# Autodesk Inventor assembly: cable-hanger-hook
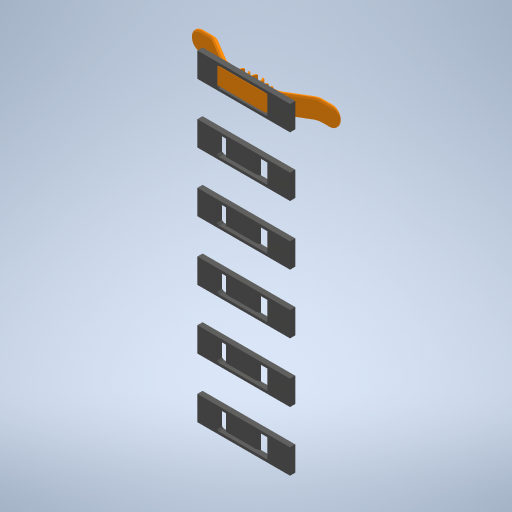
[picture p0: Inventor's stored thumbnail of the model, 512x512]
Saved by Autodesk Inventor 2023 (Build 270158030, 158C)
## iProperties
Created: 2024-09-23
Part Number: cable-hanger-hook
Document SubType Name: Assembly
Designer: Imogen Heard
Author: Imogen Heard
## Documents named in this file (3)
- C:\Users\dheard\Documents\0004-inventor\3D-CAD-main\cable-hanger\cable-hanger-hook.iam
- C:\Users\dheard\Documents\0004-inventor\3D-CAD-main\cable-hanger\cable-hanger.ipt
- C:\Users\dheard\Documents\0004-inventor\3D-CAD-main\cable-hanger\backplate-0.ipt
## Components (2 placed, 2 different names)
1. cable-hanger:1 — Flush:1
2. backplate-0:1 — Flush:1
## Relationships (1: Flush 1)
- Flush:1: cable-hanger:1 ↔ backplate-0:1
